# Autodesk Inventor assembly: Synchronous Belts Transmission4_MIR
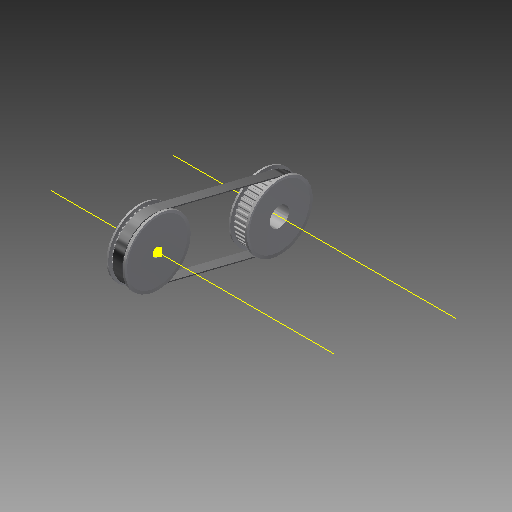
[picture p0: Inventor's stored thumbnail of the model, 512x512]
Saved by Autodesk Inventor 2019 (Build 230136000, 136)
## iProperties
Created: 2019-11-01
Part Number: Synchronous Belts Transmission4_MIR
Document SubType Name: Assembly
Designer: Mark
Author: admin
## Documents named in this file (4)
- C:\Users\Mark\Desktop\7738 Helion Engineering\7738-CAD-prep\Butterfly drive\Butterfly Drive Base\Design Accelerator\Synchronous Belts Transmission4_MIR.iam
- C:\Users\Mark\Desktop\7738 Helion Engineering\7738-CAD-prep\Butterfly drive\Butterfly Drive Base\Design Accelerator\Synchronous Belt4_MIR.ipt
- C:\Users\Mark\Desktop\7738 Helion Engineering\7738-CAD-prep\Butterfly drive\Butterfly Drive Base\Design Accelerator\Synchronous Pulley14_MIR.ipt
- C:\Users\Mark\Desktop\7738 Helion Engineering\7738-CAD-prep\Butterfly drive\Butterfly Drive Base\Design Accelerator\Synchronous Pulley24_MIR.ipt
## Components (3 placed, 3 different names)
1. Synchronous Belt4_MIR:1 — Mate:2, Mate:1, Flush:1, Mate:4, Mate:3, Flush:2
2. Synchronous Pulley14_MIR:1 — Mate:2, Mate:1, Flush:1, Rotation:1
3. Synchronous Pulley24_MIR:1 — Mate:4, Mate:3, Flush:2, Rotation:1
## Relationships (7: Flush 4, Mate 2, RelateRotation 1)
- Mate:2 [Flush]: Synchronous Belt4_MIR:1 ↔ Synchronous Pulley14_MIR:1
- Mate:1: Synchronous Belt4_MIR:1 ↔ Synchronous Pulley14_MIR:1
- Flush:1: Synchronous Belt4_MIR:1 ↔ Synchronous Pulley14_MIR:1
- Mate:4 [Flush]: Synchronous Belt4_MIR:1 ↔ Synchronous Pulley24_MIR:1
- Mate:3: Synchronous Belt4_MIR:1 ↔ Synchronous Pulley24_MIR:1
- Flush:2: Synchronous Belt4_MIR:1 ↔ Synchronous Pulley24_MIR:1
- Rotation:1 [RelateRotation] (1 ul): Synchronous Pulley14_MIR:1 ↔ Synchronous Pulley24_MIR:1
